# Autodesk Inventor assembly: Final_Assembly
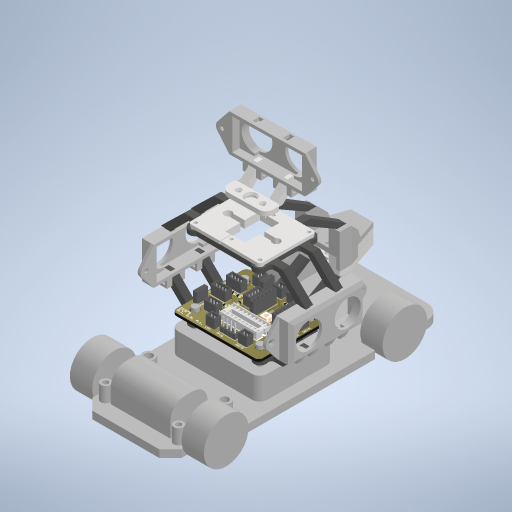
[picture p0: Inventor's stored thumbnail of the model, 512x512]
Saved by Autodesk Inventor 2024.2 (Build 282272000, 272)
## iProperties
Created: 2024-04-01
Part Number: Final_Assembly
Document SubType Name: Assembly
Designer: ringl
Author: ringl
## Documents named in this file (11)
- C:\Users\ringl\OneDrive\Uni_PC_backup\Y4S2\EE579\Assignment\EE579-Skittles\CAD\Final_Assembly.iam
- C:\Users\ringl\OneDrive\Uni_PC_backup\Y4S2\EE579\Assignment\EE579-Skittles\CAD\Bottom_Mount.ipt
- C:\Users\ringl\OneDrive\Uni_PC_backup\Y4S2\EE579\Assignment\EE579-Skittles\CAD\UltrasonicSensorMount02.ipt
- C:\Users\ringl\OneDrive\Uni_PC_backup\Y4S2\EE579\Assignment\EE579-Skittles\CAD\ServoUltrasonicMount.ipt
- C:\Users\ringl\OneDrive\Uni_PC_backup\Y4S2\EE579\Assignment\EE579-Skittles\CAD\IRMount_bottom.ipt
- C:\Users\ringl\OneDrive\Uni_PC_backup\Y4S2\EE579\Assignment\EE579-Skittles\CAD\IRMount_top.ipt
- C:\Users\ringl\OneDrive\Uni_PC_backup\Y4S2\EE579\Assignment\EE579-Skittles\CAD\ServoFullMountInsert_left.ipt
- C:\Users\ringl\OneDrive\Uni_PC_backup\Y4S2\EE579\Assignment\EE579-Skittles\CAD\ServoFullMountInsert_right.ipt
- C:\Users\ringl\OneDrive\Uni_PC_backup\Y4S2\EE579\Assignment\EE579-Skittles\CAD\Components\CarApproximation02.ipt
- C:\Users\ringl\OneDrive\Uni_PC_backup\Y4S2\EE579\Assignment\EE579-Skittles\CAD\Top_Mount.ipt
- C:\Users\ringl\OneDrive\Uni_PC_backup\Y4S2\EE579\Assignment\EE579-Skittles\CAD\PCB\EE579_Skittles_pcb\EE579_Skittles_pcb.iam
## Components (12 placed, 10 different names)
1. CarApproximation02:1 — Mate:1, Mate:2, Mate:3, Mate:24
2. Bottom_Mount:1 — Mate:1, Mate:2, Mate:3, Mate:4, Mate:5, Mate:6, Mate:7, Mate:8, Mate:9, Mate:10, Mate:11, Mate:12
3. UltrasonicSensorMount02:1 — Mate:4, Mate:5, Mate:6
4. UltrasonicSensorMount02:2 — Mate:21, Mate:22, Mate:23
5. UltrasonicSensorMount02:3 — Mate:7, Mate:8, Mate:9
6. IRMount_bottom:1 — Mate:10, Mate:11, Mate:12, Flush:1, Flush:2, Mate:13
7. IRMount_top:1 — Flush:1, Flush:2, Mate:13, Mate:14, Mate:15, Mate:16
8. Top_Mount:1 — Mate:14, Mate:15, Mate:16, Mate:17, Mate:18, Mate:19, Mate:20
9. ServoFullMountInsert_left:1 — Mate:17, Mate:18
10. ServoFullMountInsert_right:1 — Mate:19, Mate:20
11. ServoUltrasonicMount:1 — Mate:21, Mate:22, Mate:23
12. EE579_Skittles_pcb:1 [sub-assembly] — Mate:24
## Relationships (26: Mate 24, Flush 2)
- Mate:1: CarApproximation02:1 ↔ Bottom_Mount:1
- Mate:2: CarApproximation02:1 ↔ Bottom_Mount:1
- Mate:3 (2 mm): CarApproximation02:1 ↔ Bottom_Mount:1
- Mate:4: Bottom_Mount:1 ↔ UltrasonicSensorMount02:1
- Mate:5: Bottom_Mount:1 ↔ UltrasonicSensorMount02:1
- Mate:6 (0.1 mm): Bottom_Mount:1 ↔ UltrasonicSensorMount02:1
- Mate:7: Bottom_Mount:1 ↔ UltrasonicSensorMount02:3
- Mate:8: Bottom_Mount:1 ↔ UltrasonicSensorMount02:3
- Mate:9 (0.1 mm): Bottom_Mount:1 ↔ UltrasonicSensorMount02:3
- Mate:10: Bottom_Mount:1 ↔ IRMount_bottom:1
- Mate:11: Bottom_Mount:1 ↔ IRMount_bottom:1
- Mate:12: Bottom_Mount:1 ↔ IRMount_bottom:1
- Flush:1: IRMount_bottom:1 ↔ IRMount_top:1
- Flush:2: IRMount_bottom:1 ↔ IRMount_top:1
- Mate:13: IRMount_bottom:1 ↔ IRMount_top:1
- Mate:14: IRMount_top:1 ↔ Top_Mount:1
- Mate:15: IRMount_top:1 ↔ Top_Mount:1
- Mate:16: IRMount_top:1 ↔ Top_Mount:1
- Mate:17: Top_Mount:1 ↔ ServoFullMountInsert_left:1
- Mate:18: Top_Mount:1 ↔ ServoFullMountInsert_left:1
- Mate:19: Top_Mount:1 ↔ ServoFullMountInsert_right:1
- Mate:20: Top_Mount:1 ↔ ServoFullMountInsert_right:1
- Mate:21: UltrasonicSensorMount02:2 ↔ ServoUltrasonicMount:1
- Mate:22: UltrasonicSensorMount02:2 ↔ ServoUltrasonicMount:1
- Mate:23: UltrasonicSensorMount02:2 ↔ ServoUltrasonicMount:1
- Mate:24: CarApproximation02:1 ↔ EE579_Skittles_pcb:1
